# Autodesk Inventor assembly: Main Assembly
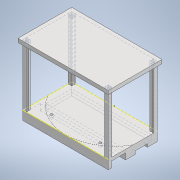
[picture p0: Inventor's stored thumbnail of the model, 180x180]
Saved by Autodesk Inventor 2022 (Build 260153000, 153)
## iProperties
Created: 2021-09-29
Part Number: Main Assembly
Document SubType Name: Assembly
Designer: andri
Author: andri
## Documents named in this file (3)
- C:\Users\andri\Downloads\Main Assembly.iam
- C:\Users\andri\Downloads\NL housing_Main.ipt
- C:\Users\andri\Downloads\NL_hosuing_Top.ipt
## Components (2 placed, 2 different names)
1. NL housing_Main:1 — Flush:1
2. NL_hosuing_Top:1 — Flush:1
## Relationships (1: Flush 1)
- Flush:1: NL housing_Main:1 ↔ NL_hosuing_Top:1
